# Autodesk Inventor assembly: 202.002.01_ZB_Rahmen_Modul
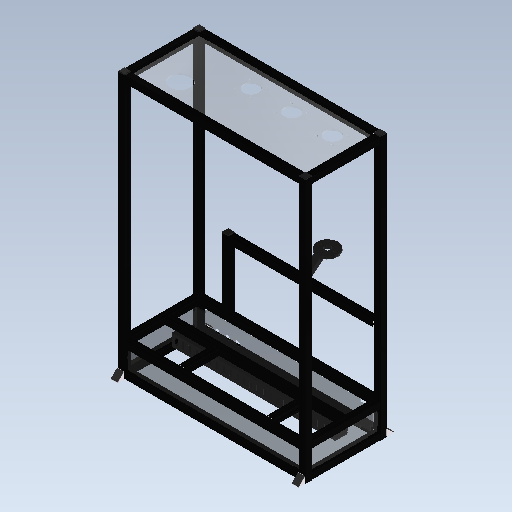
[picture p0: Inventor's stored thumbnail of the model, 512x512]
Saved by Autodesk Inventor 2022 (Build 260153000, 153)
## iProperties
Created: 2021-12-04
Part Number: 202.002.01_ZB_Rahmen_Modul
Document SubType Name: Assembly
Designer: Sebastian Seewald
Author: Sebastian Seewald
## Documents named in this file (28)
- H:\Sync-Folder\Sync\Hivemind\1-MCI-Unterlagen\Master\Semester 3\Projekt 2\011_Kartesischer_Roboter_Modul\07-CAD Files\06-Gesamtanlage\102_Rahmen_Modul\202.002.01_ZB_Rahmen_Modul.iam
- H:\Sync-Folder\Sync\Hivemind\1-MCI-Unterlagen\Master\Semester 3\Projekt 2\011_Kartesischer_Roboter_Modul\07-CAD Files\06-Gesamtanlage\102_Rahmen_Modul\502.005.01_ITEM_20x20_N1_514mm.ipt
- 502.005.01_ITEM_20x20_N1_514mm.ipt
- H:\Sync-Folder\Sync\Hivemind\1-MCI-Unterlagen\Master\Semester 3\Projekt 2\011_Kartesischer_Roboter_Modul\07-CAD Files\06-Gesamtanlage\102_Rahmen_Modul\502.002.01_ITEM_20x20_N1_200mm.ipt
- 502.002.01_ITEM_20x20_N1_200mm.ipt
- H:\Sync-Folder\Sync\Hivemind\1-MCI-Unterlagen\Master\Semester 3\Projekt 2\011_Kartesischer_Roboter_Modul\07-CAD Files\06-Gesamtanlage\102_Rahmen_Modul\502.004.01_ITEM_20x20_514mm.ipt
- 502.004.01_ITEM_20x20_514mm.ipt
- H:\Sync-Folder\Sync\Hivemind\1-MCI-Unterlagen\Master\Semester 3\Projekt 2\011_Kartesischer_Roboter_Modul\07-CAD Files\06-Gesamtanlage\102_Rahmen_Modul\502.007.01_ITEM_20x20_N1_776mm.ipt
- 502.007.01_ITEM_20x20_N1_776mm.ipt
- H:\Sync-Folder\Sync\Hivemind\1-MCI-Unterlagen\Master\Semester 3\Projekt 2\011_Kartesischer_Roboter_Modul\07-CAD Files\06-Gesamtanlage\102_Rahmen_Modul\502.001.01_ITEM_20x20_100mm.ipt
- 502.001.01_ITEM_20x20_100mm.ipt
- H:\Sync-Folder\Sync\Hivemind\1-MCI-Unterlagen\Master\Semester 3\Projekt 2\011_Kartesischer_Roboter_Modul\07-CAD Files\06-Gesamtanlage\102_Rahmen_Modul\502.003.01_ITEM_20x20_428mm.ipt
- 502.003.01_ITEM_20x20_428mm.ipt
- H:\Sync-Folder\Sync\Hivemind\1-MCI-Unterlagen\Master\Semester 3\Projekt 2\011_Kartesischer_Roboter_Modul\07-CAD Files\06-Gesamtanlage\102_Rahmen_Modul\502.008.01_ITEM_20x20_200mm.ipt
- 502.008.01_ITEM_20x20_200mm.ipt
- H:\Sync-Folder\Sync\Hivemind\1-MCI-Unterlagen\Master\Semester 3\Projekt 2\011_Kartesischer_Roboter_Modul\07-CAD Files\06-Gesamtanlage\102_Rahmen_Modul\502.009.01_ITEM_20x20_N2_514mm.ipt
- 502.009.01_ITEM_20x20_N2_514mm.ipt
- H:\Sync-Folder\Sync\Hivemind\1-MCI-Unterlagen\Master\Semester 3\Projekt 2\011_Kartesischer_Roboter_Modul\07-CAD Files\06-Gesamtanlage\102_Rahmen_Modul\502.010.01_ITEM_20x20_N2_200mm.ipt
- 502.010.01_ITEM_20x20_N2_200mm.ipt
- H:\Sync-Folder\Sync\Hivemind\1-MCI-Unterlagen\Master\Semester 3\Projekt 2\011_Kartesischer_Roboter_Modul\07-CAD Files\06-Gesamtanlage\102_Rahmen_Modul\502.011.01_Abdeckkappe_5_20x20.ipt
- H:\Sync-Folder\Sync\Hivemind\1-MCI-Unterlagen\Master\Semester 3\Projekt 2\011_Kartesischer_Roboter_Modul\07-CAD Files\06-Gesamtanlage\102_Rahmen_Modul\202.001.01_ZB_ITEM_Winkelsatz_5_20x20.iam
- H:\Sync-Folder\Sync\Hivemind\1-MCI-Unterlagen\Master\Semester 3\Projekt 2\011_Kartesischer_Roboter_Modul\07-CAD Files\06-Gesamtanlage\102_Rahmen_Modul\102.001.01_Abdeckung_Gestell_seitlich.ipt
- H:\Sync-Folder\Sync\Hivemind\1-MCI-Unterlagen\Master\Semester 3\Projekt 2\011_Kartesischer_Roboter_Modul\07-CAD Files\06-Gesamtanlage\102_Rahmen_Modul\102.002.01_Abdeckung_Gestell_front.ipt
- H:\Sync-Folder\Sync\Hivemind\1-MCI-Unterlagen\Master\Semester 3\Projekt 2\011_Kartesischer_Roboter_Modul\07-CAD Files\06-Gesamtanlage\102_Rahmen_Modul\102.003.01_Abdeckung_Gestell_hinten.ipt
- H:\Sync-Folder\Sync\Hivemind\1-MCI-Unterlagen\Master\Semester 3\Projekt 2\011_Kartesischer_Roboter_Modul\07-CAD Files\06-Gesamtanlage\102_Rahmen_Modul\102.005.01_Abdeckung_Gestell_oben.ipt
- H:\Sync-Folder\Sync\Hivemind\1-MCI-Unterlagen\Master\Semester 3\Projekt 2\011_Kartesischer_Roboter_Modul\07-CAD Files\06-Gesamtanlage\102_Rahmen_Modul\102.004.01_Lampenaufnahme.ipt
- H:\Sync-Folder\Sync\Hivemind\1-MCI-Unterlagen\Master\Semester 3\Projekt 2\011_Kartesischer_Roboter_Modul\07-CAD Files\06-Gesamtanlage\102_Rahmen_Modul\Schrauben\DIN_EN_ISO_4762_M4x16.ipt
- H:\Sync-Folder\Sync\Hivemind\1-MCI-Unterlagen\Master\Semester 3\Projekt 2\011_Kartesischer_Roboter_Modul\07-CAD Files\06-Gesamtanlage\102_Rahmen_Modul\502.016.01_Kabelkanal.ipt
## Components (38 placed, 19 different names)
1. 502.005.01_ITEM_20x20_N1_514mm:1 — Passend:1, Fluchtend:1, Passend:2, Fluchtend:2, Passend:3, Fluchtend:3, Fluchtend:8, Passend:6, Fluchtend:44, Fluchtend:51, Fluchtend:54, Passend:45
2. 502.002.01_ITEM_20x20_N1_200mm:1 — Passend:2, Fluchtend:2, Fluchtend:10, Passend:11, Fluchtend:22, Passend:25, Fluchtend:23, Passend:37, Passend:51
3. 502.002.01_ITEM_20x20_N1_200mm:2 — Passend:1, Fluchtend:1, Fluchtend:6, Fluchtend:7, Passend:5, Passend:12, Passend:49
4. 502.004.01_ITEM_20x20_514mm:1 — Passend:3, Passend:8, Fluchtend:46, Fluchtend:47, Passend:47
5. 502.006.01_ITEM_20x20_N2_776mm:2 — Fluchtend:6, Fluchtend:7, Passend:5, Passend:8, Passend:10, Fluchtend:15, Passend:14, Passend:33, Fluchtend:40, Fluchtend:46, Fluchtend:47, Fluchtend:49, Passend:43, Fluchtend:55, Fluchtend:56, Passend:48, Passend:50
6. 502.006.01_ITEM_20x20_N2_776mm:3 — Fluchtend:3, Fluchtend:34, Passend:34, Fluchtend:42, Passend:38, Fluchtend:44, Fluchtend:45, Passend:40, Fluchtend:50, Fluchtend:52, Passend:41
7. 502.006.01_ITEM_20x20_N2_776mm:4 — Fluchtend:8, Passend:6, Fluchtend:10, Fluchtend:14, Passend:29, Fluchtend:30, Passend:36, Fluchtend:35, Passend:37, Passend:39, Fluchtend:43, Fluchtend:48, Fluchtend:53, Passend:42, Passend:46, Passend:56, Fluchtend:59
8. 502.007.01_ITEM_20x20_N1_776mm:1 — Fluchtend:22, Passend:25, Fluchtend:23, Passend:26, Fluchtend:24, Passend:28, Passend:30, Fluchtend:28, Fluchtend:29, Passend:31, Fluchtend:31, Fluchtend:32, Passend:35, Fluchtend:37, Fluchtend:38, Passend:44, Fluchtend:57, Fluchtend:58, Passend:52
9. 502.002.01_ITEM_20x20_N1_200mm:3 — Fluchtend:14, Passend:11, Passend:19, Passend:26, Passend:63
10. 502.002.01_ITEM_20x20_N1_200mm:4 — Passend:10, Fluchtend:15, Passend:12, Fluchtend:16, Fluchtend:18, Passend:15, Fluchtend:19, Passend:20, Fluchtend:45
11. 502.005.01_ITEM_20x20_N1_514mm:3 — Fluchtend:16, Passend:17, Fluchtend:20, Passend:18, Fluchtend:21, Passend:38, Passend:39, Fluchtend:43
12. 502.004.01_ITEM_20x20_514mm:2 — Passend:14, Fluchtend:18, Passend:16, Passend:22, Passend:23
13. 502.001.01_ITEM_20x20_100mm:1 — Passend:17, Fluchtend:20, Passend:20
14. 502.001.01_ITEM_20x20_100mm:2 — Passend:18, Fluchtend:21, Passend:19, Passend:27
15. 502.004.01_ITEM_20x20_514mm:3 — Passend:15, Fluchtend:19, Passend:16, Passend:27, Passend:61, Passend:62
16. 502.003.01_ITEM_20x20_428mm:1 — Passend:22, Passend:24, Fluchtend:24, Passend:28, Fluchtend:25
17. 502.008.01_ITEM_20x20_200mm:1 — Passend:23, Passend:24, Fluchtend:25, Passend:58, Fluchtend:60, Fluchtend:61
18. 502.009.01_ITEM_20x20_N2_514mm:1 — Passend:30, Fluchtend:28, Fluchtend:29, Passend:55
19. 502.009.01_ITEM_20x20_N2_514mm:2 — Passend:29, Fluchtend:30, Fluchtend:48
20. 502.010.01_ITEM_20x20_N2_200mm:1 — Passend:31, Fluchtend:31, Fluchtend:32, Passend:57
21. 502.010.01_ITEM_20x20_N2_200mm:2 — Fluchtend:34, Passend:40, Fluchtend:49, Passend:53, Passend:54
22. 502.011.01_Abdeckkappe_5_20x20:1 — Passend:33, Fluchtend:40
23. 502.011.01_Abdeckkappe_5_20x20:2 — Passend:34, Fluchtend:42, Fluchtend:50
24. 502.011.01_Abdeckkappe_5_20x20:3 — Passend:35, Fluchtend:37, Fluchtend:38
25. 502.011.01_Abdeckkappe_5_20x20:4 — Passend:36, Fluchtend:35
26. 502.011.01_Abdeckkappe_5_20x20:5 — Passend:58, Fluchtend:60, Fluchtend:61
27. 202.001.01_ZB_ITEM_Winkelsatz_5_20x20:1 [sub-assembly] — Fluchtend:51, Fluchtend:52, Passend:41
28. 202.001.01_ZB_ITEM_Winkelsatz_5_20x20:2 [sub-assembly] — Fluchtend:53, Fluchtend:54, Passend:42
29. 202.001.01_ZB_ITEM_Winkelsatz_5_20x20:3 [sub-assembly] — Passend:43, Fluchtend:55, Fluchtend:56
30. 202.001.01_ZB_ITEM_Winkelsatz_5_20x20:4 [sub-assembly] — Passend:44, Fluchtend:57, Fluchtend:58
31. 102.001.01_Abdeckung_Gestell_seitlich:1 — Passend:49, Passend:50
32. 102.001.01_Abdeckung_Gestell_seitlich:2 — Passend:51, Passend:52
33. 102.002.01_Abdeckung_Gestell_front:1 — Passend:45, Passend:46
34. 102.003.01_Abdeckung_Gestell_hinten:1 — Passend:47, Passend:48
35. 102.005.01_Abdeckung_Gestell_oben:1 — Passend:53, Passend:54, Passend:55
36. 102.004.01_Lampenaufnahme:1 — Passend:56, Fluchtend:59, Passend:57, Passend:59, Passend:60
37. DIN_EN_ISO_4762_M4x16:1 — Passend:59, Passend:60
38. 502.016.01_Kabelkanal:1 — Passend:61, Passend:62, Passend:63
## Relationships (105: Mate 57, Flush 48)
- Passend:1 [Mate]: 502.005.01_ITEM_20x20_N1_514mm:1 ↔ 502.002.01_ITEM_20x20_N1_200mm:2
- Fluchtend:1 [Flush]: 502.005.01_ITEM_20x20_N1_514mm:1 ↔ 502.002.01_ITEM_20x20_N1_200mm:2
- Passend:2 [Mate]: 502.005.01_ITEM_20x20_N1_514mm:1 ↔ 502.002.01_ITEM_20x20_N1_200mm:1
- Fluchtend:2 [Flush]: 502.005.01_ITEM_20x20_N1_514mm:1 ↔ 502.002.01_ITEM_20x20_N1_200mm:1
- Passend:3 [Mate]: 502.005.01_ITEM_20x20_N1_514mm:1 ↔ 502.004.01_ITEM_20x20_514mm:1
- Fluchtend:3 [Flush]: 502.005.01_ITEM_20x20_N1_514mm:1 ↔ 502.006.01_ITEM_20x20_N2_776mm:3
- Fluchtend:6 [Flush]: 502.002.01_ITEM_20x20_N1_200mm:2 ↔ 502.006.01_ITEM_20x20_N2_776mm:2
- Fluchtend:7 [Flush]: 502.002.01_ITEM_20x20_N1_200mm:2 ↔ 502.006.01_ITEM_20x20_N2_776mm:2
- Passend:5 [Mate]: 502.002.01_ITEM_20x20_N1_200mm:2 ↔ 502.006.01_ITEM_20x20_N2_776mm:2
- Fluchtend:8 [Flush]: 502.005.01_ITEM_20x20_N1_514mm:1 ↔ 502.006.01_ITEM_20x20_N2_776mm:4
- Passend:6 [Mate]: 502.005.01_ITEM_20x20_N1_514mm:1 ↔ 502.006.01_ITEM_20x20_N2_776mm:4
- Fluchtend:10 [Flush]: 502.002.01_ITEM_20x20_N1_200mm:1 ↔ 502.006.01_ITEM_20x20_N2_776mm:4
- Passend:8 [Mate]: 502.004.01_ITEM_20x20_514mm:1 ↔ 502.006.01_ITEM_20x20_N2_776mm:2
- Fluchtend:14 [Flush]: 502.006.01_ITEM_20x20_N2_776mm:4 ↔ 502.002.01_ITEM_20x20_N1_200mm:3
- Passend:10 [Mate]: 502.006.01_ITEM_20x20_N2_776mm:2 ↔ 502.002.01_ITEM_20x20_N1_200mm:4
- Fluchtend:15 [Flush]: 502.006.01_ITEM_20x20_N2_776mm:2 ↔ 502.002.01_ITEM_20x20_N1_200mm:4
- Passend:11 [Mate] (60 mm): 502.002.01_ITEM_20x20_N1_200mm:1 ↔ 502.002.01_ITEM_20x20_N1_200mm:3
- Passend:12 [Mate] (60 mm): 502.002.01_ITEM_20x20_N1_200mm:2 ↔ 502.002.01_ITEM_20x20_N1_200mm:4
- Fluchtend:16 [Flush]: 502.002.01_ITEM_20x20_N1_200mm:4 ↔ 502.005.01_ITEM_20x20_N1_514mm:3
- Passend:14 [Mate]: 502.006.01_ITEM_20x20_N2_776mm:2 ↔ 502.004.01_ITEM_20x20_514mm:2
- Fluchtend:18 [Flush]: 502.002.01_ITEM_20x20_N1_200mm:4 ↔ 502.004.01_ITEM_20x20_514mm:2
- Passend:15 [Mate]: 502.002.01_ITEM_20x20_N1_200mm:4 ↔ 502.004.01_ITEM_20x20_514mm:3
- Fluchtend:19 [Flush]: 502.002.01_ITEM_20x20_N1_200mm:4 ↔ 502.004.01_ITEM_20x20_514mm:3
- Passend:16 [Mate] (80 mm): 502.004.01_ITEM_20x20_514mm:2 ↔ 502.004.01_ITEM_20x20_514mm:3
- Passend:17 [Mate]: 502.005.01_ITEM_20x20_N1_514mm:3 ↔ 502.001.01_ITEM_20x20_100mm:1
- Fluchtend:20 [Flush]: 502.005.01_ITEM_20x20_N1_514mm:3 ↔ 502.001.01_ITEM_20x20_100mm:1
- Passend:18 [Mate]: 502.005.01_ITEM_20x20_N1_514mm:3 ↔ 502.001.01_ITEM_20x20_100mm:2
- Fluchtend:21 [Flush]: 502.005.01_ITEM_20x20_N1_514mm:3 ↔ 502.001.01_ITEM_20x20_100mm:2
- Passend:19 [Mate] (95 mm): 502.002.01_ITEM_20x20_N1_200mm:3 ↔ 502.001.01_ITEM_20x20_100mm:2
- Passend:20 [Mate] (139 mm): 502.002.01_ITEM_20x20_N1_200mm:4 ↔ 502.001.01_ITEM_20x20_100mm:1
- Passend:22 [Mate] (180 mm): 502.004.01_ITEM_20x20_514mm:2 ↔ 502.003.01_ITEM_20x20_428mm:1
- Passend:23 [Mate]: 502.004.01_ITEM_20x20_514mm:2 ↔ 502.008.01_ITEM_20x20_200mm:1
- Passend:24 [Mate]: 502.003.01_ITEM_20x20_428mm:1 ↔ 502.008.01_ITEM_20x20_200mm:1
- Fluchtend:22 [Flush]: 502.002.01_ITEM_20x20_N1_200mm:1 ↔ 502.007.01_ITEM_20x20_N1_776mm:1
- Passend:25 [Mate]: 502.002.01_ITEM_20x20_N1_200mm:1 ↔ 502.007.01_ITEM_20x20_N1_776mm:1
- Fluchtend:23 [Flush]: 502.002.01_ITEM_20x20_N1_200mm:1 ↔ 502.007.01_ITEM_20x20_N1_776mm:1
- Passend:26 [Mate]: 502.007.01_ITEM_20x20_N1_776mm:1 ↔ 502.002.01_ITEM_20x20_N1_200mm:3
- Passend:27 [Mate]: 502.001.01_ITEM_20x20_100mm:2 ↔ 502.004.01_ITEM_20x20_514mm:3
- Fluchtend:24 [Flush]: 502.007.01_ITEM_20x20_N1_776mm:1 ↔ 502.003.01_ITEM_20x20_428mm:1
- Passend:28 [Mate]: 502.007.01_ITEM_20x20_N1_776mm:1 ↔ 502.003.01_ITEM_20x20_428mm:1
- Fluchtend:25 [Flush]: 502.003.01_ITEM_20x20_428mm:1 ↔ 502.008.01_ITEM_20x20_200mm:1
- Passend:29 [Mate]: 502.006.01_ITEM_20x20_N2_776mm:4 ↔ 502.009.01_ITEM_20x20_N2_514mm:2
- Passend:30 [Mate]: 502.007.01_ITEM_20x20_N1_776mm:1 ↔ 502.009.01_ITEM_20x20_N2_514mm:1
- Fluchtend:28 [Flush]: 502.007.01_ITEM_20x20_N1_776mm:1 ↔ 502.009.01_ITEM_20x20_N2_514mm:1
- Fluchtend:29 [Flush]: 502.007.01_ITEM_20x20_N1_776mm:1 ↔ 502.009.01_ITEM_20x20_N2_514mm:1
- Fluchtend:30 [Flush]: 502.006.01_ITEM_20x20_N2_776mm:4 ↔ 502.009.01_ITEM_20x20_N2_514mm:2
- Passend:31 [Mate]: 502.007.01_ITEM_20x20_N1_776mm:1 ↔ 502.010.01_ITEM_20x20_N2_200mm:1
- Fluchtend:31 [Flush]: 502.007.01_ITEM_20x20_N1_776mm:1 ↔ 502.010.01_ITEM_20x20_N2_200mm:1
- Fluchtend:32 [Flush]: 502.007.01_ITEM_20x20_N1_776mm:1 ↔ 502.010.01_ITEM_20x20_N2_200mm:1
- Fluchtend:34 [Flush]: 502.006.01_ITEM_20x20_N2_776mm:3 ↔ 502.010.01_ITEM_20x20_N2_200mm:2
- Passend:33 [Mate]: 502.006.01_ITEM_20x20_N2_776mm:2 ↔ 502.011.01_Abdeckkappe_5_20x20:1
- Passend:34 [Mate]: 502.006.01_ITEM_20x20_N2_776mm:3 ↔ 502.011.01_Abdeckkappe_5_20x20:2
- Passend:35 [Mate]: 502.007.01_ITEM_20x20_N1_776mm:1 ↔ 502.011.01_Abdeckkappe_5_20x20:3
- Passend:36 [Mate]: 502.006.01_ITEM_20x20_N2_776mm:4 ↔ 502.011.01_Abdeckkappe_5_20x20:4
- Fluchtend:35 [Flush]: 502.006.01_ITEM_20x20_N2_776mm:4 ↔ 502.011.01_Abdeckkappe_5_20x20:4
- Fluchtend:37 [Flush]: 502.007.01_ITEM_20x20_N1_776mm:1 ↔ 502.011.01_Abdeckkappe_5_20x20:3
- Fluchtend:38 [Flush]: 502.007.01_ITEM_20x20_N1_776mm:1 ↔ 502.011.01_Abdeckkappe_5_20x20:3
- Fluchtend:40 [Flush]: 502.006.01_ITEM_20x20_N2_776mm:2 ↔ 502.011.01_Abdeckkappe_5_20x20:1
- Fluchtend:42 [Flush]: 502.006.01_ITEM_20x20_N2_776mm:3 ↔ 502.011.01_Abdeckkappe_5_20x20:2
- Passend:37 [Mate]: 502.002.01_ITEM_20x20_N1_200mm:1 ↔ 502.006.01_ITEM_20x20_N2_776mm:4
- Passend:38 [Mate]: 502.006.01_ITEM_20x20_N2_776mm:3 ↔ 502.005.01_ITEM_20x20_N1_514mm:3
- Passend:39 [Mate]: 502.006.01_ITEM_20x20_N2_776mm:4 ↔ 502.005.01_ITEM_20x20_N1_514mm:3
- Fluchtend:43 [Flush]: 502.006.01_ITEM_20x20_N2_776mm:4 ↔ 502.005.01_ITEM_20x20_N1_514mm:3
- Fluchtend:44 [Flush]: 502.005.01_ITEM_20x20_N1_514mm:1 ↔ 502.006.01_ITEM_20x20_N2_776mm:3
- Fluchtend:45 [Flush]: 502.006.01_ITEM_20x20_N2_776mm:3 ↔ 502.002.01_ITEM_20x20_N1_200mm:4
- Fluchtend:46 [Flush]: 502.004.01_ITEM_20x20_514mm:1 ↔ 502.006.01_ITEM_20x20_N2_776mm:2
- Fluchtend:47 [Flush]: 502.004.01_ITEM_20x20_514mm:1 ↔ 502.006.01_ITEM_20x20_N2_776mm:2
- Fluchtend:48 [Flush]: 502.006.01_ITEM_20x20_N2_776mm:4 ↔ 502.009.01_ITEM_20x20_N2_514mm:2
- Passend:40 [Mate]: 502.006.01_ITEM_20x20_N2_776mm:3 ↔ 502.010.01_ITEM_20x20_N2_200mm:2
- Fluchtend:49 [Flush]: 502.006.01_ITEM_20x20_N2_776mm:2 ↔ 502.010.01_ITEM_20x20_N2_200mm:2
- Fluchtend:50 [Flush]: 502.006.01_ITEM_20x20_N2_776mm:3 ↔ 502.011.01_Abdeckkappe_5_20x20:2
- Fluchtend:51 [Flush]: 502.005.01_ITEM_20x20_N1_514mm:1 ↔ 202.001.01_ZB_ITEM_Winkelsatz_5_20x20:1
- Fluchtend:52 [Flush]: 502.006.01_ITEM_20x20_N2_776mm:3 ↔ 202.001.01_ZB_ITEM_Winkelsatz_5_20x20:1
- Passend:41 [Mate]: 502.006.01_ITEM_20x20_N2_776mm:3 ↔ 202.001.01_ZB_ITEM_Winkelsatz_5_20x20:1
- Fluchtend:53 [Flush]: 502.006.01_ITEM_20x20_N2_776mm:4 ↔ 202.001.01_ZB_ITEM_Winkelsatz_5_20x20:2
- Fluchtend:54 [Flush]: 502.005.01_ITEM_20x20_N1_514mm:1 ↔ 202.001.01_ZB_ITEM_Winkelsatz_5_20x20:2
- Passend:42 [Mate]: 502.006.01_ITEM_20x20_N2_776mm:4 ↔ 202.001.01_ZB_ITEM_Winkelsatz_5_20x20:2
- Passend:43 [Mate]: 502.006.01_ITEM_20x20_N2_776mm:2 ↔ 202.001.01_ZB_ITEM_Winkelsatz_5_20x20:3
- Fluchtend:55 [Flush]: 502.006.01_ITEM_20x20_N2_776mm:2 ↔ 202.001.01_ZB_ITEM_Winkelsatz_5_20x20:3
- Fluchtend:56 [Flush]: 502.006.01_ITEM_20x20_N2_776mm:2 ↔ 202.001.01_ZB_ITEM_Winkelsatz_5_20x20:3
- Passend:44 [Mate]: 502.007.01_ITEM_20x20_N1_776mm:1 ↔ 202.001.01_ZB_ITEM_Winkelsatz_5_20x20:4
- Fluchtend:57 [Flush]: 502.007.01_ITEM_20x20_N1_776mm:1 ↔ 202.001.01_ZB_ITEM_Winkelsatz_5_20x20:4
- Fluchtend:58 [Flush]: 502.007.01_ITEM_20x20_N1_776mm:1 ↔ 202.001.01_ZB_ITEM_Winkelsatz_5_20x20:4
- Passend:45 [Mate]: 502.005.01_ITEM_20x20_N1_514mm:1 ↔ 102.002.01_Abdeckung_Gestell_front:1
- Passend:46 [Mate]: 502.006.01_ITEM_20x20_N2_776mm:4 ↔ 102.002.01_Abdeckung_Gestell_front:1
- Passend:47 [Mate]: 502.004.01_ITEM_20x20_514mm:1 ↔ 102.003.01_Abdeckung_Gestell_hinten:1
- Passend:48 [Mate]: 502.006.01_ITEM_20x20_N2_776mm:2 ↔ 102.003.01_Abdeckung_Gestell_hinten:1
- Passend:49 [Mate]: 502.002.01_ITEM_20x20_N1_200mm:2 ↔ 102.001.01_Abdeckung_Gestell_seitlich:1
- Passend:50 [Mate]: 502.006.01_ITEM_20x20_N2_776mm:2 ↔ 102.001.01_Abdeckung_Gestell_seitlich:1
- Passend:51 [Mate]: 502.002.01_ITEM_20x20_N1_200mm:1 ↔ 102.001.01_Abdeckung_Gestell_seitlich:2
- Passend:52 [Mate]: 502.007.01_ITEM_20x20_N1_776mm:1 ↔ 102.001.01_Abdeckung_Gestell_seitlich:2
- Passend:53 [Mate]: 502.010.01_ITEM_20x20_N2_200mm:2 ↔ 102.005.01_Abdeckung_Gestell_oben:1
- Passend:54 [Mate]: 502.010.01_ITEM_20x20_N2_200mm:2 ↔ 102.005.01_Abdeckung_Gestell_oben:1
- Passend:55 [Mate]: 502.009.01_ITEM_20x20_N2_514mm:1 ↔ 102.005.01_Abdeckung_Gestell_oben:1
- Passend:56 [Mate]: 502.006.01_ITEM_20x20_N2_776mm:4 ↔ 102.004.01_Lampenaufnahme:1
- Fluchtend:59 [Flush]: 502.006.01_ITEM_20x20_N2_776mm:4 ↔ 102.004.01_Lampenaufnahme:1
- Passend:57 [Mate] (195.5 mm): 502.010.01_ITEM_20x20_N2_200mm:1 ↔ 102.004.01_Lampenaufnahme:1
- Passend:58 [Mate]: 502.008.01_ITEM_20x20_200mm:1 ↔ 502.011.01_Abdeckkappe_5_20x20:5
- Fluchtend:60 [Flush]: 502.008.01_ITEM_20x20_200mm:1 ↔ 502.011.01_Abdeckkappe_5_20x20:5
- Fluchtend:61 [Flush]: 502.008.01_ITEM_20x20_200mm:1 ↔ 502.011.01_Abdeckkappe_5_20x20:5
- Passend:59 [Mate]: 102.004.01_Lampenaufnahme:1 ↔ DIN_EN_ISO_4762_M4x16:1
- Passend:60 [Mate]: 102.004.01_Lampenaufnahme:1 ↔ DIN_EN_ISO_4762_M4x16:1
- Passend:61 [Mate]: 502.004.01_ITEM_20x20_514mm:3 ↔ 502.016.01_Kabelkanal:1
- Passend:62 [Mate] (-10 mm): 502.004.01_ITEM_20x20_514mm:3 ↔ 502.016.01_Kabelkanal:1
- Passend:63 [Mate] (5 mm): 502.002.01_ITEM_20x20_N1_200mm:3 ↔ 502.016.01_Kabelkanal:1
